# Autodesk Inventor assembly: Assembly1
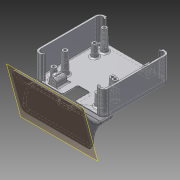
[picture p0: Inventor's stored thumbnail of the model, 180x180]
Saved by Autodesk Inventor 2013 (Build 170138000, 138)
## iProperties
Created: 2013-10-08
Part Number: Assembly1
Document SubType Name: Assembly
Designer: md
Author: md
## Documents named in this file (3)
- X:\Projects\hexasense\enclosure\sense_board_v2\Assembly1.iam
- X:\PROJECTS\HEXASENSE\ENCLOSURE\SENSE_BOARD_V2\Gehaeuse.ipt
- X:\Projects\hexasense\enclosure\sense_board_v2\Staender.ipt
## Components (2 placed, 2 different names)
1. Gehaeuse:1 — Flush:1, Mate:1, Mate:2
2. STAENDER:1 — Flush:1, Mate:1, Mate:2
## Relationships (3: Mate 2, Flush 1)
- Flush:1: Gehaeuse:1 ↔ STAENDER:1
- Mate:1: Gehaeuse:1 ↔ STAENDER:1
- Mate:2: Gehaeuse:1 ↔ STAENDER:1
